# Autodesk Inventor assembly: 2016-02-10-RobotV16
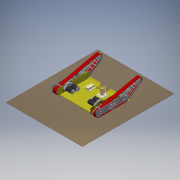
[picture p0: Inventor's stored thumbnail of the model, 180x180]
Saved by Autodesk Inventor 2016 SP1 (Build 200210100, 210)
## iProperties
Created: 2016-02-10
Part Number: 2016-02-10-RobotV16
Document SubType Name: Assembly
Designer: steele
Author: steele
## Documents named in this file (8)
- C:\snobotics\CAD-Development\robSteele\SnoBotics2016\2016-02-08-RhinoTrackWithSheetBase\2016-02-10-RobotV16.iam
- C:\snobotics\CAD-Development\robSteele\SnoBotics2016\RhinoTrackDriveModule\am-3322+RhinoTrackDriveModule.iam
- C:\snobotics\CAD-Development\robSteele\SnoBotics2016\RhinoBottomFloorOptions\SheetBottomFloorV01.ipt
- C:\snobotics\CAD-Development\robSteele\SnoBotics2016\RhinoTrackDriveModule\am-3322+RhinoTrackDriveModule_MIR13.iam
- C:\snobotics\CAD-Development\robSteele\SnoBotics2016\RhinoBottomFloorOptions\Floor.ipt
- C:\snobotics\CAD-Development\robSteele\SnoBotics2016\DraftOfBoulder.ipt
- C:\snobotics\CAD-Development\robSteele\SnoBotics2016\2016-05-05-ShooterPrototype\SupportPlateMotorMountV01.ipt
- C:\snobotics\CAD-Development\robSteele\SnoBotics2016\2016-05-05-ShooterPrototype\SupportPlateWithPostOnlyV01.ipt
## Components (7 placed, 7 different names)
1. am-3322+RhinoTrackDriveModule:1 [sub-assembly] — Mate:1, Flush:1, Flush:2, Mate:4
2. SheetBottomFloorV01:1 — Mate:1, Flush:1, Flush:2, Mate:2, Mate:3, Flush:6, Flush:8, Mate:6, Mate:7, Mate:8, Mate:9, Flush:10
3. am-3322+RhinoTrackDriveModule_MIR13:1 [sub-assembly]
4. Floor:1 — Mate:2, Mate:3, Mate:4, Flush:7, Mate:5
5. DraftOfBoulder:1 — Flush:6, Flush:7, Mate:5
6. SupportPlateMotorMountV01:1 — Mate:6, Mate:8, Flush:9, Flush:10
7. SupportPlateWithPostOnlyV01:1 — Mate:7, Mate:9, Flush:9
## Relationships (16: Mate 9, Flush 7)
- Mate:1: am-3322+RhinoTrackDriveModule:1 ↔ SheetBottomFloorV01:1
- Flush:1: am-3322+RhinoTrackDriveModule:1 ↔ SheetBottomFloorV01:1
- Flush:2 (4.7625 mm): am-3322+RhinoTrackDriveModule:1 ↔ SheetBottomFloorV01:1
- Mate:2: SheetBottomFloorV01:1 ↔ Floor:1
- Mate:3: SheetBottomFloorV01:1 ↔ Floor:1
- Mate:4: am-3322+RhinoTrackDriveModule:1 ↔ Floor:1
- Flush:6: SheetBottomFloorV01:1 ↔ DraftOfBoulder:1
- Flush:7 (127 mm): Floor:1 ↔ DraftOfBoulder:1
- Mate:5 (-381 mm): Floor:1 ↔ DraftOfBoulder:1
- Flush:8: SheetBottomFloorV01:1
- Mate:6: SheetBottomFloorV01:1 ↔ SupportPlateMotorMountV01:1
- Mate:7: SheetBottomFloorV01:1 ↔ SupportPlateWithPostOnlyV01:1
- Mate:8 (101.6 mm): SheetBottomFloorV01:1 ↔ SupportPlateMotorMountV01:1
- Mate:9 (304.8 mm): SheetBottomFloorV01:1 ↔ SupportPlateWithPostOnlyV01:1
- Flush:9: SupportPlateMotorMountV01:1 ↔ SupportPlateWithPostOnlyV01:1
- Flush:10: SheetBottomFloorV01:1 ↔ SupportPlateMotorMountV01:1
